# Autodesk Inventor assembly: Prototype Assembly
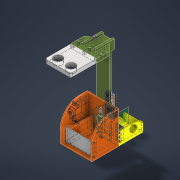
[picture p0: Inventor's stored thumbnail of the model, 180x180]
Saved by Autodesk Inventor 2022 (Build 260153000, 153)
## iProperties
Created: 2021-05-30
Part Number: Prototype Assembly
Document SubType Name: Assembly
Designer: sidsa
Author: sidsa
## Documents named in this file (13)
- D:\CODING\auto-dispenser\Inventor\Prototype Assembly.iam
- D:\CODING\auto-dispenser\Inventor\Hand Sanitizer (prototype).ipt
- D:\CODING\auto-dispenser\Inventor\PreCAD\ServoMotor.ipt
- D:\CODING\auto-dispenser\Inventor\Vertical Beam Prototype.ipt
- D:\CODING\auto-dispenser\Inventor\PreCAD\hc-sr04.ipt
- D:\CODING\auto-dispenser\Inventor\PreCAD\Arduino_NANO_CH340.ipt
- D:\CODING\auto-dispenser\Inventor\PreCAD\solar_panel.ipt
- D:\CODING\auto-dispenser\Inventor\Base.ipt
- D:\CODING\auto-dispenser\Inventor\Sliding Plate.ipt
- D:\CODING\auto-dispenser\Inventor\Sliding Pin.ipt
- D:\CODING\auto-dispenser\Inventor\Electronics Tray.ipt
- C:\Users\hasht\Documents\Ultrasonic Mount.ipt
- C:\Users\hasht\Documents\Ultrasonic Locking Pin.ipt
## Components (14 placed, 12 different names)
1. Hand Sanitizer (prototype):1 — Flush:4
2. ServoMotor:1 — Flush:6, Mate:9
3. Vertical Beam Prototype:1 — Flush:7, Mate:10, Mate:11, Mate:12, Mate:13, Mate:14, Mate:15, Flush:9, Flush:10, Flush:11, Flush:12
4. hc-sr04:1
5. Arduino_NANO_CH340:1
6. solar_panel:1 — Mate:15, Flush:9
7. Base:1 — Flush:4, Flush:5, Flush:6, Mate:9, Flush:7, Flush:8, Mate:10, Mate:11
8. Sliding Plate:1 — Flush:5
9. Sliding Pin:1 — Flush:8
10. Electronics Tray:1 — Mate:12, Mate:13, Mate:14
11. Ultrasonic Mount:1 — Flush:10, Flush:11, Flush:12
12. Ultrasonic Locking Pin:1
13. Ultrasonic Locking Pin:2
14. Ultrasonic Locking Pin:3
## Relationships (16: Flush 9, Mate 7)
- Flush:4: Hand Sanitizer (prototype):1 ↔ Base:1
- Flush:5: Base:1 ↔ Sliding Plate:1
- Flush:6: ServoMotor:1 ↔ Base:1
- Mate:9: ServoMotor:1 ↔ Base:1
- Flush:7: Vertical Beam Prototype:1 ↔ Base:1
- Flush:8: Base:1 ↔ Sliding Pin:1
- Mate:10: Vertical Beam Prototype:1 ↔ Base:1
- Mate:11: Vertical Beam Prototype:1 ↔ Base:1
- Mate:12: Vertical Beam Prototype:1 ↔ Electronics Tray:1
- Mate:13: Vertical Beam Prototype:1 ↔ Electronics Tray:1
- Mate:14: Vertical Beam Prototype:1 ↔ Electronics Tray:1
- Mate:15: Vertical Beam Prototype:1 ↔ solar_panel:1
- Flush:9: Vertical Beam Prototype:1 ↔ solar_panel:1
- Flush:10: Vertical Beam Prototype:1 ↔ Ultrasonic Mount:1
- Flush:11: Vertical Beam Prototype:1 ↔ Ultrasonic Mount:1
- Flush:12: Vertical Beam Prototype:1 ↔ Ultrasonic Mount:1
